# Autodesk Inventor assembly: tail_p3
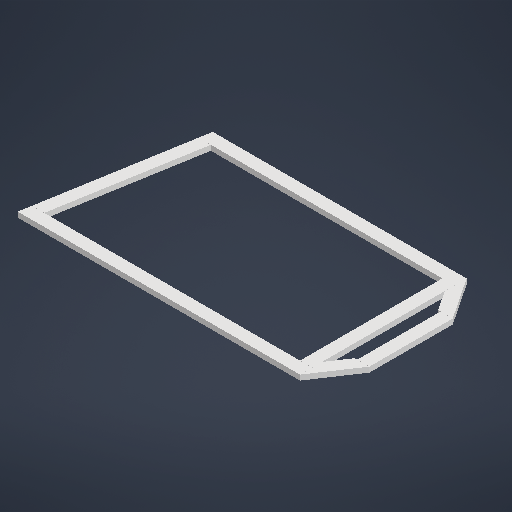
[picture p0: Inventor's stored thumbnail of the model, 512x512]
Saved by Autodesk Inventor 2027.1 (Build 311270010, 270A)
## iProperties
Created: 2026-09-01
Part Number: tail_p3
Document SubType Name: Assembly
Designer: jorda
Author: jorda
## Documents named in this file (7)
- C:\Users\jorda\OneDrive\Documents\GitHub\USC-ASME-TigerBurn-2026\CAD\Tail\tail_p4.iam
- C:\Users\jorda\OneDrive\Documents\GitHub\USC-ASME-TigerBurn-2026\CAD\Tail\S_2x4x48.76.ipt
- C:\Users\jorda\OneDrive\Documents\GitHub\USC-ASME-TigerBurn-2026\CAD\Tail\2x4x41.ipt
- C:\Users\jorda\OneDrive\Documents\GitHub\USC-ASME-TigerBurn-2026\CAD\Tail\S_2x4x84.ipt
- C:\Users\jorda\OneDrive\Documents\GitHub\USC-ASME-TigerBurn-2026\CAD\Tail\S_2x4x73.75.ipt
- C:\Users\jorda\OneDrive\Documents\GitHub\USC-ASME-TigerBurn-2026\CAD\Tail\2x4x24.ipt
- C:\Users\jorda\OneDrive\Documents\GitHub\USC-ASME-TigerBurn-2026\CAD\Tail\S_2x4x14.42.ipt
## Components (7 placed, 6 different names)
1. S_2x4x48.76:1 — Mate:6, Flush:5, Flush:6, Mate:7, Flush:7, Mate:8
2. S_2x4x84:1 — Mate:6, Flush:5, Flush:6, Mate:12
3. S_2x4x73.75:1 — Mate:7, Flush:7, Mate:8, Mate:9, Flush:8, Flush:9, Mate:11, Flush:10
4. 2x4x41:1 — Mate:9, Flush:8, Flush:9, Mate:10, Flush:11
5. 2x4x24:1 — Mate:13, Flush:12, Mate:14
6. S_2x4x14.42:1 — Mate:10, Mate:11, Flush:10
7. S_2x4x14.42:2 — Mate:12, Flush:11, Mate:13, Flush:12, Mate:14
## Relationships (17: Mate 9, Flush 8)
- Mate:6: S_2x4x48.76:1 ↔ S_2x4x84:1
- Flush:5: S_2x4x48.76:1 ↔ S_2x4x84:1
- Flush:6: S_2x4x48.76:1 ↔ S_2x4x84:1
- Mate:7: S_2x4x48.76:1 ↔ S_2x4x73.75:1
- Flush:7: S_2x4x48.76:1 ↔ S_2x4x73.75:1
- Mate:8: S_2x4x48.76:1 ↔ S_2x4x73.75:1
- Mate:9: S_2x4x73.75:1 ↔ 2x4x41:1
- Flush:8: S_2x4x73.75:1 ↔ 2x4x41:1
- Flush:9: S_2x4x73.75:1 ↔ 2x4x41:1
- Mate:10: 2x4x41:1 ↔ S_2x4x14.42:1
- Mate:11: S_2x4x73.75:1 ↔ S_2x4x14.42:1
- Flush:10: S_2x4x73.75:1 ↔ S_2x4x14.42:1
- Mate:12: S_2x4x84:1 ↔ S_2x4x14.42:2
- Flush:11: 2x4x41:1 ↔ S_2x4x14.42:2
- Mate:13: 2x4x24:1 ↔ S_2x4x14.42:2
- Flush:12: 2x4x24:1 ↔ S_2x4x14.42:2
- Mate:14: 2x4x24:1 ↔ S_2x4x14.42:2
